# Autodesk Inventor assembly: WheelieBar Blue Alliance
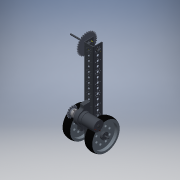
[picture p0: Inventor's stored thumbnail of the model, 180x180]
Saved by Autodesk Inventor 2016 (Build 200138000, 138)
## iProperties
Created: 2015-12-14
Part Number: WheelieBar Blue Alliance
Document SubType Name: Assembly
Designer: tbloo
Author: tbloo
## Documents named in this file (15)
- C:\Users\TimB\Documents\GitHub\phi_robotics\3d-models\FTC_Tetrix_KOP_Block_Party\Tim Bloot Designs\JAr JaR Bot\WheelieBar Red Alliance.iam
- C:\Users\TimB\Documents\GitHub\phi_robotics\3d-models\FTC_Tetrix_KOP_Block_Party\Tetrix_Kit_FTC\Autodesk Inventor Files\tetrix_axle.ipt
- C:\Users\TimB\Documents\GitHub\phi_robotics\3d-models\FTC_Tetrix_KOP_Block_Party\Tetrix_Kit_FTC\Autodesk Inventor Files\tetrix_axle_lock.iam
- C:\Users\TimB\Documents\GitHub\phi_robotics\3d-models\FTC_Tetrix_KOP_Block_Party\Tetrix_Kit_FTC\Autodesk Inventor Files\tetrix_screw.ipt
- C:\Users\TimB\Documents\GitHub\phi_robotics\3d-models\FTC_Tetrix_KOP_Block_Party\Tetrix_Kit_FTC\Autodesk Inventor Files\tetrix_bushing.ipt
- C:\Users\TimB\Documents\GitHub\phi_robotics\3d-models\FTC_Tetrix_KOP_Block_Party\Tetrix_Kit_FTC\Autodesk Inventor Files\tetrix_axle_spacer-small.ipt
- C:\Users\TimB\Documents\GitHub\phi_robotics\3d-models\FTC_Tetrix_KOP_Block_Party\Tetrix_Kit_FTC\Autodesk Inventor Files\tetrix_motor_mount-old.ipt
- C:\Users\TimB\Documents\GitHub\phi_robotics\3d-models\FTC_Tetrix_KOP_Block_Party\Tetrix_Kit_FTC\Autodesk Inventor Files\tetrix_c_channel-4.ipt
- C:\Users\TimB\Documents\GitHub\phi_robotics\3d-models\FTC_Tetrix_KOP_Block_Party\Tetrix_Kit_FTC\Autodesk Inventor Files\tetrix_chain_gear-16t.ipt
- C:\Users\TimB\Documents\GitHub\phi_robotics\3d-models\FTC_Tetrix_KOP_Block_Party\Tetrix_Kit_FTC\Autodesk Inventor Files\tetrix_chain_gear-32t.ipt
- C:\Users\TimB\Documents\GitHub\phi_robotics\3d-models\FTC_Tetrix_KOP_Block_Party\Tetrix_Kit_FTC\Autodesk Inventor Files\tetrix_739092_2012.iam
- C:\Users\TimB\Documents\GitHub\phi_robotics\3d-models\FTC_Tetrix_KOP_Block_Party\Tetrix_Kit_FTC\Autodesk Inventor Files\tetrix_wheel.ipt
- C:\Users\TimB\Documents\GitHub\phi_robotics\3d-models\FTC_Tetrix_KOP_Block_Party\Tetrix_Kit_FTC\Autodesk Inventor Files\tetrix_axle_spacer-big.ipt
- C:\Users\TimB\Documents\GitHub\phi_robotics\3d-models\FTC_Tetrix_KOP_Block_Party\Tetrix_Kit_FTC\Autodesk Inventor Files\tetrix_motor.iam
- C:\Users\TimB\Documents\GitHub\phi_robotics\3d-models\FTC_Tetrix_KOP_Block_Party\Tetrix_Kit_FTC\Autodesk Inventor Files\tetrix_maxle_lock.iam
## Components (26 placed, 14 different names)
1. tetrix_c_channel-4:1 — Rigid:1, Rigid:2, Rigid:6, Rotational:2, Rotational:6, Rigid:22
2. tetrix_axle_lock:1 [sub-assembly] — Rigid:10, Rigid:13
3. tetrix_axle:1 — Rigid:12, Rigid:18
4. tetrix_axle:2 — Rigid:8
5. tetrix_chain_gear-32t:1 — Rigid:2, Rigid:3, Rigid:4, Rigid:5
6. tetrix_chain_gear-16t:1 — Rigid:11, Rigid:14, Rigid:15, Rigid:16
7. tetrix_739092_2012:1 [sub-assembly] — Rigid:7, Rigid:8
8. tetrix_motor_mount-old:1 — Rigid:22, Rotational:8
9. tetrix_axle_lock:2 [sub-assembly] — Rigid:1
10. tetrix_screw:1 — Rigid:3
11. tetrix_screw:2 — Rigid:4
12. tetrix_axle_spacer-small:1 — Rigid:5
13. tetrix_bushing:1 — Rigid:6, Rigid:7
14. tetrix_wheel:1 — Rigid:10, Rigid:12
15. tetrix_wheel:2 — Rigid:17, Rigid:18
16. tetrix_axle_lock:3 [sub-assembly] — Rigid:11, Rigid:13
17. tetrix_screw:3 — Rigid:14
18. tetrix_screw:4 — Rigid:15
19. tetrix_axle_spacer-small:2 — Rigid:16, Rotational:7
20. tetrix_bushing:2 — Rotational:4, Rotational:6
21. tetrix_bushing:3 — Rotational:2, Rotational:7
22. tetrix_axle_lock:4 [sub-assembly] — Rigid:17
23. tetrix_axle_spacer-big:1 — Rotational:4
24. tetrix_motor:2 [sub-assembly] — Rigid:21, Rotational:8
25. tetrix_chain_gear-16t:2
26. tetrix_maxle_lock:1 [sub-assembly] — Rigid:21
## Relationships (25: WeldJoint 20, RevoluteJoint 5)
- Rigid:1 [WeldJoint]: tetrix_c_channel-4:1 ↔ tetrix_axle_lock:2
- Rigid:2 [WeldJoint]: tetrix_c_channel-4:1 ↔ tetrix_chain_gear-32t:1
- Rigid:3 [WeldJoint]: tetrix_chain_gear-32t:1 ↔ tetrix_screw:1
- Rigid:4 [WeldJoint]: tetrix_chain_gear-32t:1 ↔ tetrix_screw:2
- Rigid:5 [WeldJoint]: tetrix_chain_gear-32t:1 ↔ tetrix_axle_spacer-small:1
- Rigid:6 [WeldJoint]: tetrix_c_channel-4:1 ↔ tetrix_bushing:1
- Rigid:7 [WeldJoint]: tetrix_739092_2012:1 ↔ tetrix_bushing:1
- Rigid:8 [WeldJoint]: tetrix_axle:2 ↔ tetrix_739092_2012:1
- Rigid:10 [WeldJoint]: tetrix_axle_lock:1 ↔ tetrix_wheel:1
- Rigid:11 [WeldJoint]: tetrix_chain_gear-16t:1 ↔ tetrix_axle_lock:3
- Rigid:12 [WeldJoint]: tetrix_axle:1 ↔ tetrix_wheel:1
- Rigid:13 [WeldJoint]: tetrix_axle_lock:1 ↔ tetrix_axle_lock:3
- Rigid:14 [WeldJoint]: tetrix_chain_gear-16t:1 ↔ tetrix_screw:3
- Rigid:15 [WeldJoint]: tetrix_chain_gear-16t:1 ↔ tetrix_screw:4
- Rigid:16 [WeldJoint]: tetrix_chain_gear-16t:1 ↔ tetrix_axle_spacer-small:2
- Rotational:2 [RevoluteJoint]: tetrix_c_channel-4:1 ↔ tetrix_bushing:3
- Rigid:17 [WeldJoint]: tetrix_wheel:2 ↔ tetrix_axle_lock:4
- Rotational:4 [RevoluteJoint]: tetrix_bushing:2 ↔ tetrix_axle_spacer-big:1
- Rigid:18 [WeldJoint] (-25.5 mm): tetrix_axle:1 ↔ tetrix_wheel:2
- Rotational:6 [RevoluteJoint]: tetrix_c_channel-4:1 ↔ tetrix_bushing:2
- Rotational:7 [RevoluteJoint]: tetrix_axle_spacer-small:2 ↔ tetrix_bushing:3
- [WeldJoint]: tetrix_chain_gear-16t:2 ↔ tetrix_maxle_lock:1
- Rigid:21 [WeldJoint] (-23 mm): tetrix_motor:2 ↔ tetrix_maxle_lock:1
- Rigid:22 [WeldJoint]: tetrix_c_channel-4:1 ↔ tetrix_motor_mount-old:1
- Rotational:8 [RevoluteJoint]: tetrix_motor_mount-old:1 ↔ tetrix_motor:2
